# Autodesk Inventor assembly: printedWheel
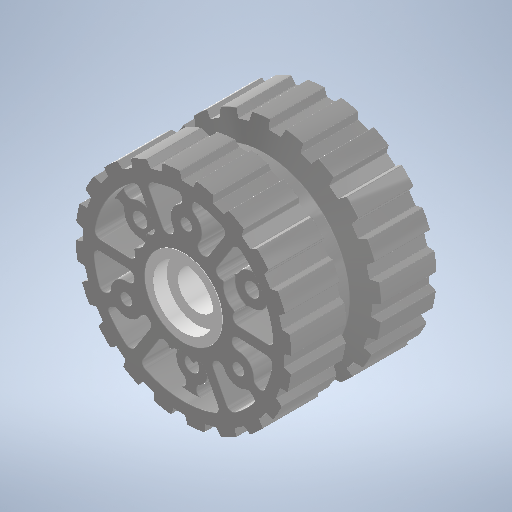
[picture p0: Inventor's stored thumbnail of the model, 512x512]
Saved by Autodesk Inventor 2025 (Build 290162000, 162)
## iProperties
Created: 2024-10-28
Part Number: printedWheel
Document SubType Name: Assembly
Designer: derm
Author: derm
## Documents named in this file (3)
- C:\Users\derm\Desktop\puppycat\printedWheel.iam
- C:\Users\derm\Desktop\puppycat\am-3298a 20 tooth Molded Tank Pulley Half Rev4\am-3298a 20 tooth Molded Tank Pulley Half Rev4.ipt
- C:\Users\derm\Desktop\puppycat\am3298_bearing_adapter.ipt
## Components (4 placed, 2 different names)
1. am-3298a 20 tooth Molded Tank Pulley Half Rev4:1
2. am-3298a 20 tooth Molded Tank Pulley Half Rev4:2
3. am3298_bearing_adapter:1
4. am3298_bearing_adapter:2
## Relationships (6: Mate 6)
- [Mate]: am-3298a 20 tooth Molded Tank Pulley Half Rev4:1 ↔ am-3298a 20 tooth Molded Tank Pulley Half Rev4:2
- [Mate]: am-3298a 20 tooth Molded Tank Pulley Half Rev4:1 ↔ am-3298a 20 tooth Molded Tank Pulley Half Rev4:2
- [Mate]: am-3298a 20 tooth Molded Tank Pulley Half Rev4:1 ↔ am-3298a 20 tooth Molded Tank Pulley Half Rev4:2
- [Mate]: am-3298a 20 tooth Molded Tank Pulley Half Rev4:2 ↔ am3298_bearing_adapter:1
- [Mate]: am-3298a 20 tooth Molded Tank Pulley Half Rev4:1 ↔ am3298_bearing_adapter:2
- [Mate]: am-3298a 20 tooth Molded Tank Pulley Half Rev4:1 ↔ am3298_bearing_adapter:2
## Named parameters: d57_d17_d10 = 0 mm, d60_d20_d13 = 0 mm, d61_d21_d14 = 0 mm, d64_d24_d0 = 0 mm, d65_d25_d1 = 0 mm, d66_d26_d2 = 0 mm
